# Autodesk Inventor assembly: UmlenkrolleHalterDoppeltAngle
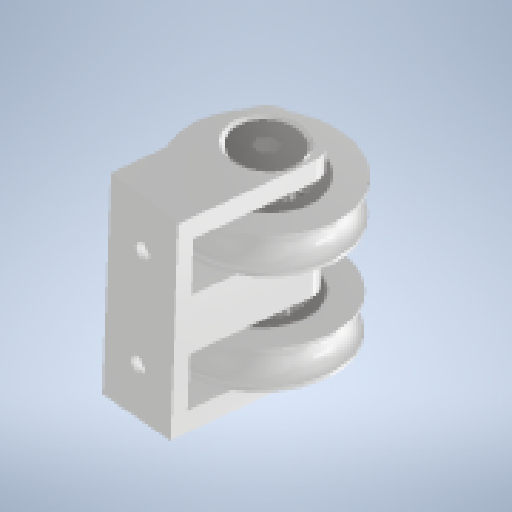
[picture p0: Inventor's stored thumbnail of the model, 512x512]
Saved by Autodesk Inventor 2025 (Build 290162010, 162A)
## iProperties
Created: 2024-11-19
Part Number: UmlenkrolleHalterDoppeltAngle
Document SubType Name: Assembly
Designer: Admin
Mass: 13.7211 g
Surface Area: 66.6118 cm^2
Volume: 4.83602 cm^3
Density: 2.83726 g/cm^3
Author: Admin
## Documents named in this file (5)
- C:\Users\Admin\Documents\Inventor\Krandemonstrator\UmlenkrolleHalterDoppeltAngle.iam
- C:\Users\Admin\Documents\Inventor\Krandemonstrator\Umlenkrolle.iam
- C:\Users\Admin\Documents\Inventor\Content Center Files\R2025\de-DE\AS 1237 (2.1)\AS 1237 - 4.ipt
- C:\Users\Admin\Documents\Inventor\Krandemonstrator\HalterUmlenkrolleDPLAngle.ipt
- C:\Users\Admin\Documents\Inventor\Content Center Files\R2025\de-DE\DIN 7991(2)\DIN 7991 - M4x12.ipt
## Components (9 placed, 4 different names)
1. Umlenkrolle:1 [sub-assembly] — Drehbar:9
2. AS 1237 (2.1) 4:1 — Drehbar:11
3. AS 1237 (2.1) 4:2 — Drehbar:7, Drehbar:12
4. AS 1237 (2.1) 4:3 — Drehbar:5, Drehbar:9
5. Umlenkrolle:2 [sub-assembly] — Drehbar:12
6. HalterUmlenkrolleDPLAngle:1 — Drehbar:5, Drehbar:7, Drehbar:10, Drehbar:11, Starr:1, Starr:2
7. DIN 7991 M4x12:1 — Starr:1
8. DIN 7991 M4x12:2 — Starr:2
9. AS 1237 (2.1) 4:4 — Drehbar:10
## Relationships (8: RevoluteJoint 6, WeldJoint 2)
- Drehbar:5 [RevoluteJoint]: AS 1237 (2.1) 4:3 ↔ HalterUmlenkrolleDPLAngle:1
- Drehbar:7 [RevoluteJoint]: AS 1237 (2.1) 4:2 ↔ HalterUmlenkrolleDPLAngle:1
- Drehbar:9 [RevoluteJoint]: Umlenkrolle:1 ↔ AS 1237 (2.1) 4:3
- Drehbar:10 [RevoluteJoint]: HalterUmlenkrolleDPLAngle:1 ↔ AS 1237 (2.1) 4:4
- Drehbar:11 [RevoluteJoint]: AS 1237 (2.1) 4:1 ↔ HalterUmlenkrolleDPLAngle:1
- Drehbar:12 [RevoluteJoint]: AS 1237 (2.1) 4:2 ↔ Umlenkrolle:2
- Starr:1 [WeldJoint]: HalterUmlenkrolleDPLAngle:1 ↔ DIN 7991 M4x12:1
- Starr:2 [WeldJoint]: HalterUmlenkrolleDPLAngle:1 ↔ DIN 7991 M4x12:2
